# Autodesk Inventor assembly: 42146-01
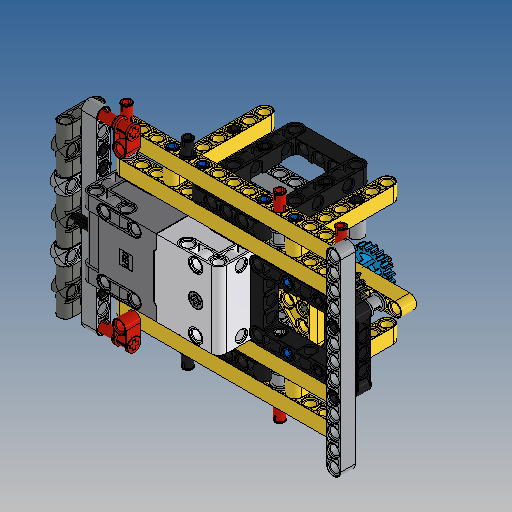
[picture p0: Inventor's stored thumbnail of the model, 512x512]
Saved by Autodesk Inventor 2025 (Build 290162010, 162A)
## iProperties
Created: 2024-11-11
Part Number: 42146-01
Material: Generisch
Document SubType Name: Assembly
Designer: hp.muther
Author: hp.muther
## Documents named in this file (26)
- D:\Inventor\Projekte\Muther\LEGO Technic\LEGO Technik - Raupenkran LR 13000 (42146)\42146-01-01.iam
- D:\Inventor\Projekte\Muther\LEGO Technic\LEGO Pieces\69730 - MOTOR, NR. 15.ipt
- D:\Inventor\Projekte\Muther\LEGO Technic\LEGO Pieces\Pin's\2780-Black.ipt
- D:\Inventor\Projekte\Muther\LEGO Technic\LEGO Pieces\Lochbalken\32278-Yellow.ipt
- D:\Inventor\Projekte\Muther\LEGO Technic\LEGO Pieces\Pin's\11214-Red.ipt
- D:\Inventor\Projekte\Muther\LEGO Technic\LEGO Pieces\Pin's\32054-LtBluishGray.ipt
- D:\Inventor\Projekte\Muther\LEGO Technic\LEGO Pieces\Pin's\6558-Blue.ipt
- D:\Inventor\Projekte\Muther\LEGO Technic\LEGO Pieces\Rahmen, T-Stücke\64179-Black.ipt
- D:\Inventor\Projekte\Muther\LEGO Technic\LEGO Pieces\Lochbalken\41239-LtBluishGray.ipt
- D:\Inventor\Projekte\Muther\LEGO Technic\LEGO Pieces\Lochbalken\32316-LtBluishGray.ipt
- D:\Inventor\Projekte\Muther\LEGO Technic\LEGO Pieces\Pin's\43093-Blue.ipt
- D:\Inventor\Projekte\Muther\LEGO Technic\LEGO Pieces\Verbindungselemente\15461-Black.ipt
- D:\Inventor\Projekte\Muther\LEGO Technic\LEGO Pieces\Rahmen, T-Stücke\99773-Yellow.ipt
- D:\Inventor\Projekte\Muther\LEGO Technic\LEGO Pieces\Achsen\87083-DkBluishGray.ipt
- D:\Inventor\Projekte\Muther\LEGO Technic\LEGO Pieces\Zahnrad\10928-DkBluishGray.ipt
- D:\Inventor\Projekte\Muther\LEGO Technic\LEGO Pieces\Zahnrad\69779-DkAzure.ipt
- D:\Inventor\Projekte\Muther\LEGO Technic\LEGO Pieces\Zahnrad\69778-Blue.ipt
- D:\Inventor\Projekte\Muther\LEGO Technic\LEGO Pieces\Achsen\99008-Tan.ipt
- D:\Inventor\Projekte\Muther\LEGO Technic\LEGO Pieces\Achsen\32209-DkBluishGray.ipt
- D:\Inventor\Projekte\Muther\LEGO Technic\LEGO Pieces\Zahnrad\3648-DkBluishGray.ipt
- D:\Inventor\Projekte\Muther\LEGO Technic\LEGO Pieces\Rund\18654-Red.ipt
- D:\Inventor\Projekte\Muther\LEGO Technic\LEGO Pieces\Lochbalken\32524-Yellow.ipt
- D:\Inventor\Projekte\Muther\LEGO Technic\LEGO Pieces\Lochbalken\40490-LtBluishGray.ipt
- D:\Inventor\Projekte\Muther\LEGO Technic\LEGO Pieces\Verbindungselemente\6536-Red.ipt
- D:\Inventor\Projekte\Muther\LEGO Technic\LEGO Pieces\Verbindungselemente\39793-LtBluishGray.ipt
- D:\Inventor\Projekte\Muther\LEGO Technic\LEGO Pieces\Verbindungselemente\48989-LtBluishGray.ipt
## Components (105 placed, 25 different names)
1. 69730 - MOTOR, NR. 15:1 — Einfügen:1, Einfügen:2, Einfügen:3, Einfügen:4, Einfügen:5, Einfügen:6, Einfügen:11, Einfügen:29, Einfügen:44, Passend:7, Passend:59, Einfügen:59, Passend:13, Passend:60, Einfügen:93
2. 2780-Black:1 — Einfügen:2
3. 2780-Black:2 — Einfügen:1, Passend:3
4. 2780-Black:3 — Einfügen:6, Passend:81
5. 2780-Black:4 — Einfügen:5
6. 2780-Black:5 — Einfügen:3, Passend:1
7. 2780-Black:6 — Einfügen:4
8. 32278-Yellow:1 — Einfügen:10, Einfügen:11, Passend:1, Einfügen:12, Einfügen:13, Einfügen:14, Einfügen:15, Einfügen:16, Einfügen:17, Einfügen:18, Einfügen:83
9. 11214-Red:1 — Einfügen:9, Einfügen:85
10. 11214-Red:2 — Einfügen:7
11. 11214-Red:3 — Einfügen:8, Passend:79
12. 32054-LtBluishGray:1 — Einfügen:9, Einfügen:10
13. 32054-LtBluishGray:2 — Einfügen:7, Einfügen:12
14. 32054-LtBluishGray:3 — Einfügen:8, Einfügen:13, Passend:2
15. 6558-Blue:1 — Einfügen:16, Passend:75
16. 6558-Blue:2 — Einfügen:14, Passend:77
17. 6558-Blue:3 — Einfügen:15
18. 6558-Blue:4 — Einfügen:17, Passend:76
19. 64179-Black:1 — Einfügen:18, Passend:2, Einfügen:32, Passend:4, Einfügen:43, Passend:8, Einfügen:60, Passend:14
20. 32278-Yellow:2 — Einfügen:29, Passend:3, Einfügen:82
21. 11214-Red:4 — Einfügen:87
22. 11214-Red:5
23. 11214-Red:6 — Passend:80
24. 32054-LtBluishGray:4
25. 32054-LtBluishGray:5
26. 32054-LtBluishGray:6
27. 6558-Blue:5
28. 6558-Blue:6 — Passend:73
29. 6558-Blue:7 — Passend:72
30. 6558-Blue:8 — Passend:74
31. 2780-Black:7 — Einfügen:31, Einfügen:32
32. 2780-Black:8 — Einfügen:30, Passend:4
33. 41239-LtBluishGray:1 — Einfügen:30, Einfügen:31
34. 32316-LtBluishGray:1 — Einfügen:34, Passend:5, Einfügen:36, Einfügen:37, Einfügen:44
35. 32054-LtBluishGray:7 — Einfügen:33, Einfügen:35
36. 43093-Blue:1 — Einfügen:33, Passend:78
37. 2780-Black:9 — Einfügen:36, Passend:7
38. 15461-Black:1 — Einfügen:34, Passend:5, Einfügen:35
39. 2780-Black:10 — Einfügen:37
40. 32316-LtBluishGray:2 — Einfügen:39, Einfügen:43
41. 32054-LtBluishGray:8
42. 43093-Blue:2 — Einfügen:67
43. 2780-Black:11 — Passend:8
44. 15461-Black:2 — Einfügen:39
45. 2780-Black:12
46. 99773-Yellow:1 — Einfügen:45, Passend:9, Einfügen:49, Einfügen:66
47. 99773-Yellow:2 — Einfügen:45, Passend:9, Einfügen:46, Einfügen:47, Einfügen:48, Einfügen:60
48. 43093-Blue:3 — Einfügen:47, Passend:14
49. 43093-Blue:4 — Einfügen:46
50. 87083-DkBluishGray:1 — Einfügen:48, Passend:10
51. 10928-DkBluishGray:1 — Einfügen:50, Drehung:4
52. 69779-DkAzure:1 — Einfügen:49, Passend:10, Einfügen:50, Drehung:1
53. 69778-Blue:1 — Einfügen:57, Passend:59, Drehung:1, Drehung:2
54. 99008-Tan:1 — Einfügen:57, Passend:60, Zanräder fixiert
55. 99773-Yellow:3 — Einfügen:65
56. 99773-Yellow:4 — Einfügen:54, Einfügen:59
57. 43093-Blue:5
58. 43093-Blue:6 — Passend:13
59. 87083-DkBluishGray:2 — Einfügen:54
60. 10928-DkBluishGray:2 — Drehung:3
61. 69779-DkAzure:2 — Drehung:2
62. 32209-DkBluishGray:1 — Einfügen:61, Passend:15, Einfügen:66, Passend:68, Passend:69
63. 3648-DkBluishGray:1 — Einfügen:62, Passend:15, Drehung:4
64. 18654-Red:1 — Einfügen:61, Einfügen:62
65. 32209-DkBluishGray:2 — Einfügen:65, Passend:63, Passend:66
66. 3648-DkBluishGray:2 — Drehung:3
67. 18654-Red:2
68. 32278-Yellow:3 — Einfügen:67, Passend:62, Passend:67, Passend:78, Zanräder fixiert
69. 69779-DkAzure:3 — Passend:67, Passend:68, Passend:69
70. 69779-DkAzure:4 — Passend:62, Passend:63, Passend:66
71. 64179-Black:2 — Einfügen:70, Einfügen:71, Einfügen:82, Passend:72
72. 32524-Yellow:1 — Einfügen:69, Passend:73
73. 32524-Yellow:2 — Einfügen:68, Passend:74
74. 40490-LtBluishGray:1 — Einfügen:72, Passend:70, Einfügen:73, Einfügen:74
75. 2780-Black:13 — Einfügen:71, Einfügen:72
76. 2780-Black:14 — Einfügen:69, Einfügen:74
77. 2780-Black:15 — Einfügen:70, Passend:70
78. 2780-Black:16 — Einfügen:68, Einfügen:73
79. 64179-Black:3 — Einfügen:83, Passend:75
80. 32524-Yellow:3 — Einfügen:76, Passend:77
81. 32524-Yellow:4 — Passend:76
82. 40490-LtBluishGray:2
83. 2780-Black:17
84. 2780-Black:18 — Einfügen:76
85. 2780-Black:19
86. 2780-Black:20
87. 32278-Yellow:4 — Einfügen:84, Einfügen:85, Passend:79
88. 2780-Black:21 — Einfügen:84
89. 32278-Yellow:5 — Einfügen:87, Passend:80
90. 2780-Black:22
91. 11214-Red:7 — Einfügen:94, Passend:84
92. 2780-Black:23 — Einfügen:90, Einfügen:100
93. 2780-Black:24 — Einfügen:91
94. 2780-Black:25 — Einfügen:89
95. 2780-Black:26 — Einfügen:88, Passend:90
96. 2780-Black:27 — Einfügen:92
97. 41239-LtBluishGray:2 — Einfügen:88, Einfügen:89, Einfügen:90, Einfügen:91, Einfügen:92, Einfügen:93, Passend:81, Passend:82, Winkel:2, Passend:83, Passend:85, Passend:84, Winkel:3
98. 6536-Red:1 — Einfügen:94, Winkel:3, Passend:85
99. 11214-Red:8 — Passend:82
100. 6536-Red:2 — Winkel:2, Passend:83
101. 39793-LtBluishGray:1 — Einfügen:97, Einfügen:99, Passend:86, Passend:87
102. 39793-LtBluishGray:2 — Einfügen:96, Passend:88, Passend:90
103. 48989-LtBluishGray:1 — Einfügen:96, Einfügen:97, Passend:87, Passend:88
104. 39793-LtBluishGray:3 — Einfügen:100, Passend:89
105. 48989-LtBluishGray:2 — Einfügen:99, Passend:86, Passend:89
## Relationships (151: Insert 99, Mate 45, RelateRotation 4, Angle 3)
- Winkel:3 [Angle] (0 deg): 41239-LtBluishGray:2 ↔ 6536-Red:1
- Winkel:2 [Angle] (0 deg): 41239-LtBluishGray:2 ↔ 6536-Red:2
- Passend:83 [Mate] (8 mm): 41239-LtBluishGray:2 ↔ 6536-Red:2
- Passend:85 [Mate] (8 mm): 41239-LtBluishGray:2 ↔ 6536-Red:1
- Drehung:1 [RelateRotation] (0.6 ul): 69779-DkAzure:1 ↔ 69778-Blue:1
- Drehung:2 [RelateRotation] (0.6 ul): 69778-Blue:1 ↔ 69779-DkAzure:2
- Drehung:3 [RelateRotation] (3 ul): 10928-DkBluishGray:2 ↔ 3648-DkBluishGray:2
- Drehung:4 [RelateRotation] (3 ul): 10928-DkBluishGray:1 ↔ 3648-DkBluishGray:1
- Zanräder fixiert [Angle] (0 deg): 99008-Tan:1 ↔ 32278-Yellow:3
- Passend:80 [Mate]: 11214-Red:6 ↔ 32278-Yellow:5
- Einfügen:1 [Insert]: 69730 - MOTOR, NR. 15:1 ↔ 2780-Black:2
- Einfügen:2 [Insert]: 69730 - MOTOR, NR. 15:1 ↔ 2780-Black:1
- Einfügen:3 [Insert]: 69730 - MOTOR, NR. 15:1 ↔ 2780-Black:5
- Einfügen:4 [Insert]: 69730 - MOTOR, NR. 15:1 ↔ 2780-Black:6
- Einfügen:5 [Insert]: 69730 - MOTOR, NR. 15:1 ↔ 2780-Black:4
- Einfügen:6 [Insert]: 69730 - MOTOR, NR. 15:1 ↔ 2780-Black:3
- Einfügen:7 [Insert]: 11214-Red:2 ↔ 32054-LtBluishGray:2
- Einfügen:8 [Insert]: 11214-Red:3 ↔ 32054-LtBluishGray:3
- Einfügen:9 [Insert]: 11214-Red:1 ↔ 32054-LtBluishGray:1
- Einfügen:10 [Insert]: 32278-Yellow:1 ↔ 32054-LtBluishGray:1
- Einfügen:11 [Insert]: 69730 - MOTOR, NR. 15:1 ↔ 32278-Yellow:1
- Passend:1 [Mate]: 2780-Black:5 ↔ 32278-Yellow:1
- Einfügen:12 [Insert]: 32278-Yellow:1 ↔ 32054-LtBluishGray:2
- Einfügen:13 [Insert]: 32278-Yellow:1 ↔ 32054-LtBluishGray:3
- Einfügen:14 [Insert]: 32278-Yellow:1 ↔ 6558-Blue:2
- Einfügen:15 [Insert]: 32278-Yellow:1 ↔ 6558-Blue:3
- Einfügen:16 [Insert]: 32278-Yellow:1 ↔ 6558-Blue:1
- Einfügen:17 [Insert]: 32278-Yellow:1 ↔ 6558-Blue:4
- Einfügen:18 [Insert]: 32278-Yellow:1 ↔ 64179-Black:1
- Passend:2 [Mate]: 32054-LtBluishGray:3 ↔ 64179-Black:1
- [Insert]: 11214-Red:5 ↔ 32054-LtBluishGray:5
- [Insert]: 11214-Red:6 ↔ 32054-LtBluishGray:6
- [Insert]: 11214-Red:4 ↔ 32054-LtBluishGray:4
- [Insert]: 32278-Yellow:2 ↔ 32054-LtBluishGray:4
- [Insert]: 32278-Yellow:2 ↔ 32054-LtBluishGray:5
- [Insert]: 32278-Yellow:2 ↔ 32054-LtBluishGray:6
- [Insert]: 32278-Yellow:2 ↔ 6558-Blue:6
- [Insert]: 32278-Yellow:2 ↔ 6558-Blue:7
- [Insert]: 32278-Yellow:2 ↔ 6558-Blue:5
- [Insert]: 32278-Yellow:2 ↔ 6558-Blue:8
- Einfügen:29 [Insert]: 69730 - MOTOR, NR. 15:1 ↔ 32278-Yellow:2
- Passend:3 [Mate]: 2780-Black:2 ↔ 32278-Yellow:2
- Einfügen:30 [Insert]: 2780-Black:8 ↔ 41239-LtBluishGray:1
- Einfügen:31 [Insert]: 2780-Black:7 ↔ 41239-LtBluishGray:1
- Einfügen:32 [Insert]: 64179-Black:1 ↔ 2780-Black:7
- Passend:4 [Mate]: 64179-Black:1 ↔ 2780-Black:8
- Einfügen:33 [Insert]: 32054-LtBluishGray:7 ↔ 43093-Blue:1
- Einfügen:34 [Insert]: 32316-LtBluishGray:1 ↔ 15461-Black:1
- Passend:5 [Mate]: 32316-LtBluishGray:1 ↔ 15461-Black:1
- Einfügen:35 [Insert]: 32054-LtBluishGray:7 ↔ 15461-Black:1
- Einfügen:36 [Insert]: 32316-LtBluishGray:1 ↔ 2780-Black:9
- Einfügen:37 [Insert]: 32316-LtBluishGray:1 ↔ 2780-Black:10
- [Insert]: 32054-LtBluishGray:8 ↔ 43093-Blue:2
- Einfügen:39 [Insert]: 32316-LtBluishGray:2 ↔ 15461-Black:2
- [Mate]: 32316-LtBluishGray:2 ↔ 15461-Black:2
- [Insert]: 32054-LtBluishGray:8 ↔ 15461-Black:2
- [Insert]: 32316-LtBluishGray:2 ↔ 2780-Black:11
- [Insert]: 32316-LtBluishGray:2 ↔ 2780-Black:12
- Einfügen:43 [Insert]: 64179-Black:1 ↔ 32316-LtBluishGray:2
- Einfügen:44 [Insert]: 69730 - MOTOR, NR. 15:1 ↔ 32316-LtBluishGray:1
- Passend:7 [Mate]: 69730 - MOTOR, NR. 15:1 ↔ 2780-Black:9
- Passend:8 [Mate]: 64179-Black:1 ↔ 2780-Black:11
- Einfügen:45 [Insert]: 99773-Yellow:1 ↔ 99773-Yellow:2
- Passend:9 [Mate]: 99773-Yellow:1 ↔ 99773-Yellow:2
- Einfügen:46 [Insert]: 99773-Yellow:2 ↔ 43093-Blue:4
- Einfügen:47 [Insert]: 99773-Yellow:2 ↔ 43093-Blue:3
- Einfügen:48 [Insert]: 99773-Yellow:2 ↔ 87083-DkBluishGray:1
- Einfügen:49 [Insert]: 99773-Yellow:1 ↔ 69779-DkAzure:1
- Passend:10 [Mate]: 87083-DkBluishGray:1 ↔ 69779-DkAzure:1
- Einfügen:50 [Insert]: 10928-DkBluishGray:1 ↔ 69779-DkAzure:1
- [Insert]: 99773-Yellow:3 ↔ 99773-Yellow:4
- [Mate]: 99773-Yellow:3 ↔ 99773-Yellow:4
- [Insert]: 99773-Yellow:4 ↔ 43093-Blue:6
- [Insert]: 99773-Yellow:4 ↔ 43093-Blue:5
- Einfügen:54 [Insert]: 99773-Yellow:4 ↔ 87083-DkBluishGray:2
- [Insert]: 99773-Yellow:3 ↔ 69779-DkAzure:2
- [Mate]: 87083-DkBluishGray:2 ↔ 69779-DkAzure:2
- [Insert]: 10928-DkBluishGray:2 ↔ 69779-DkAzure:2
- Einfügen:57 [Insert]: 69778-Blue:1 ↔ 99008-Tan:1
- Passend:59 [Mate]: 69730 - MOTOR, NR. 15:1 ↔ 69778-Blue:1
- Einfügen:59 [Insert]: 69730 - MOTOR, NR. 15:1 ↔ 99773-Yellow:4
- Passend:13 [Mate]: 69730 - MOTOR, NR. 15:1 ↔ 43093-Blue:6
- Einfügen:60 [Insert]: 64179-Black:1 ↔ 99773-Yellow:2
- Passend:14 [Mate]: 64179-Black:1 ↔ 43093-Blue:3
- Einfügen:61 [Insert]: 32209-DkBluishGray:1 ↔ 18654-Red:1
- Einfügen:62 [Insert]: 3648-DkBluishGray:1 ↔ 18654-Red:1
- Passend:15 [Mate]: 32209-DkBluishGray:1 ↔ 3648-DkBluishGray:1
- [Insert]: 32209-DkBluishGray:2 ↔ 18654-Red:2
- [Insert]: 3648-DkBluishGray:2 ↔ 18654-Red:2
- [Mate]: 32209-DkBluishGray:2 ↔ 3648-DkBluishGray:2
- Einfügen:65 [Insert]: 99773-Yellow:3 ↔ 32209-DkBluishGray:2
- Einfügen:66 [Insert]: 99773-Yellow:1 ↔ 32209-DkBluishGray:1
- Einfügen:67 [Insert]: 43093-Blue:2 ↔ 32278-Yellow:3
- Passend:60 [Mate]: 69730 - MOTOR, NR. 15:1 ↔ 99008-Tan:1
- Passend:62 [Mate]: 32278-Yellow:3 ↔ 69779-DkAzure:4
- Passend:63 [Mate]: 32209-DkBluishGray:2 ↔ 69779-DkAzure:4
- Passend:66 [Mate]: 32209-DkBluishGray:2 ↔ 69779-DkAzure:4
- Passend:67 [Mate]: 32278-Yellow:3 ↔ 69779-DkAzure:3
- Passend:68 [Mate]: 32209-DkBluishGray:1 ↔ 69779-DkAzure:3
- Passend:69 [Mate]: 32209-DkBluishGray:1 ↔ 69779-DkAzure:3
- Einfügen:68 [Insert]: 32524-Yellow:2 ↔ 2780-Black:16
- Einfügen:69 [Insert]: 32524-Yellow:1 ↔ 2780-Black:14
- Einfügen:70 [Insert]: 64179-Black:2 ↔ 2780-Black:15
- Einfügen:71 [Insert]: 64179-Black:2 ↔ 2780-Black:13
- Einfügen:72 [Insert]: 40490-LtBluishGray:1 ↔ 2780-Black:13
- Passend:70 [Mate]: 40490-LtBluishGray:1 ↔ 2780-Black:15
- Einfügen:73 [Insert]: 40490-LtBluishGray:1 ↔ 2780-Black:16
- Einfügen:74 [Insert]: 40490-LtBluishGray:1 ↔ 2780-Black:14
- [Insert]: 32524-Yellow:4 ↔ 2780-Black:20
- Einfügen:76 [Insert]: 32524-Yellow:3 ↔ 2780-Black:18
- [Insert]: 64179-Black:3 ↔ 2780-Black:19
- [Insert]: 64179-Black:3 ↔ 2780-Black:17
- [Insert]: 40490-LtBluishGray:2 ↔ 2780-Black:17
- [Mate]: 40490-LtBluishGray:2 ↔ 2780-Black:19
- [Insert]: 40490-LtBluishGray:2 ↔ 2780-Black:20
- [Insert]: 40490-LtBluishGray:2 ↔ 2780-Black:18
- Einfügen:82 [Insert]: 32278-Yellow:2 ↔ 64179-Black:2
- Passend:72 [Mate]: 6558-Blue:7 ↔ 64179-Black:2
- Passend:73 [Mate]: 6558-Blue:6 ↔ 32524-Yellow:1
- Passend:74 [Mate]: 6558-Blue:8 ↔ 32524-Yellow:2
- Einfügen:83 [Insert]: 32278-Yellow:1 ↔ 64179-Black:3
- Passend:75 [Mate]: 6558-Blue:1 ↔ 64179-Black:3
- Passend:76 [Mate]: 6558-Blue:4 ↔ 32524-Yellow:4
- Passend:77 [Mate]: 6558-Blue:2 ↔ 32524-Yellow:3
- Passend:78 [Mate]: 43093-Blue:1 ↔ 32278-Yellow:3
- Einfügen:84 [Insert]: 32278-Yellow:4 ↔ 2780-Black:21
- Einfügen:85 [Insert]: 11214-Red:1 ↔ 32278-Yellow:4
- Passend:79 [Mate]: 11214-Red:3 ↔ 32278-Yellow:4
- [Insert]: 32278-Yellow:5 ↔ 2780-Black:22
- Einfügen:87 [Insert]: 11214-Red:4 ↔ 32278-Yellow:5
- Einfügen:88 [Insert]: 2780-Black:26 ↔ 41239-LtBluishGray:2
- Einfügen:89 [Insert]: 2780-Black:25 ↔ 41239-LtBluishGray:2
- Einfügen:90 [Insert]: 2780-Black:23 ↔ 41239-LtBluishGray:2
- Einfügen:91 [Insert]: 2780-Black:24 ↔ 41239-LtBluishGray:2
- Einfügen:92 [Insert]: 2780-Black:27 ↔ 41239-LtBluishGray:2
- Einfügen:93 [Insert]: 69730 - MOTOR, NR. 15:1 ↔ 41239-LtBluishGray:2
- Passend:81 [Mate]: 2780-Black:3 ↔ 41239-LtBluishGray:2
- Einfügen:94 [Insert]: 11214-Red:7 ↔ 6536-Red:1
- [Insert]: 11214-Red:8 ↔ 6536-Red:2
- Passend:82 [Mate]: 41239-LtBluishGray:2 ↔ 11214-Red:8
- Passend:84 [Mate]: 11214-Red:7 ↔ 41239-LtBluishGray:2
- Einfügen:96 [Insert]: 39793-LtBluishGray:2 ↔ 48989-LtBluishGray:1
- Einfügen:97 [Insert]: 39793-LtBluishGray:1 ↔ 48989-LtBluishGray:1
- [Insert]: 39793-LtBluishGray:3 ↔ 48989-LtBluishGray:2
- Einfügen:99 [Insert]: 39793-LtBluishGray:1 ↔ 48989-LtBluishGray:2
- Einfügen:100 [Insert]: 2780-Black:23 ↔ 39793-LtBluishGray:3
- Passend:86 [Mate]: 39793-LtBluishGray:1 ↔ 48989-LtBluishGray:2
- Passend:87 [Mate]: 39793-LtBluishGray:1 ↔ 48989-LtBluishGray:1
- Passend:88 [Mate]: 39793-LtBluishGray:2 ↔ 48989-LtBluishGray:1
- Passend:89 [Mate]: 39793-LtBluishGray:3 ↔ 48989-LtBluishGray:2
- Passend:90 [Mate]: 2780-Black:26 ↔ 39793-LtBluishGray:2
## Named parameters: d21_d6 = 0 mm, d22_d7 = 0 mm, d23_d8 = 0 mm, d24_d9 = 0 mm, d25_d17 = 0 mm, d26_d18 = 0 mm, d28_d13 = 0 mm, d29_d14 = 0 mm, d30_d15 = 0 mm, d31_d16 = 0 mm, d44_d38 = 0 mm, d45_d39 = 0 mm, d46_d40 = 0 mm, d47_d41 = 0 mm, d48_d42 = 0 mm, d49_d43 = 0 mm, d62_d54 = 0 mm, d63_d55 = 0 mm, d64_d56 = 0 mm, d65_d57 = 0 mm, d66_d58 = 0 mm, d67_d59 = 0 mm, d68_d60 = 0 mm, d69_d61 = 0 mm, d79_d76 = 0 mm, d80_d77 = 0 mm, d81_d78 = 0 mm, d103_d95 = 0 mm, d104_d96 = 0 mm, d105_d97 = 0 mm, d106_d98 = 0 mm, d107_d99 = 0 mm, d108_d100 = 0 mm, d109_d101 = 0 mm, d110_d102 = 0 mm, d127_d124 = 0 mm, d139_d138 = 0 mm, d148_d147 = 0 mm
